# Autodesk Inventor assembly: Probe-clamp-v1
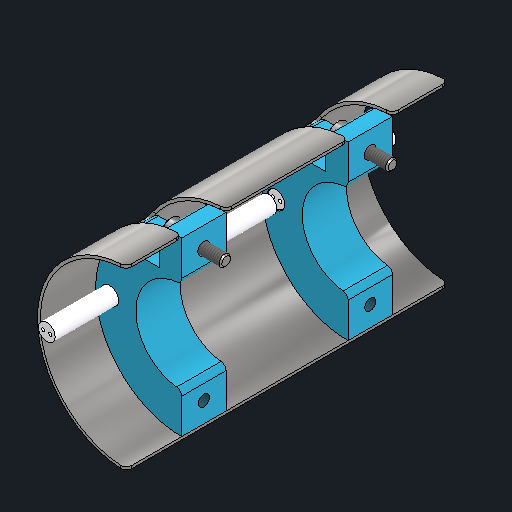
[picture p0: Inventor's stored thumbnail of the model, 512x512]
Saved by Autodesk Inventor 2026 (Build 300175050, 175E)
## iProperties
Created: 2024-06-05
Part Number: Probe-clamp-v1
Document SubType Name: Assembly
Designer: kuzmin
Author: kuzmin
## Documents named in this file (6)
- C:\Users\queez\Dropbox\Drawings\PIHTI\PALP\Probe-clamp-v1.iam
- C:\Users\queez\Dropbox\Drawings\PIHTI\PALP\WireHolderRing\WireHolderRing-ID16.4.ipt
- C:\Users\queez\Dropbox\Drawings\PIHTI\PALP\WireHolderRing.ipt
- C:\Users\queez\Dropbox\Drawings\PIHTI\ContentCenter\Fastners\M2x8-SHCS.ipt
- C:\Users\queez\Dropbox\Drawings\PIHTI\PALP\LP-screen-sheet-metal.ipt
- C:\Users\queez\Dropbox\Drawings\PIHTI\ContentCenter\Ceramics\Ceramic-tube-two-holes-phi3x0.5.ipt
## Components (8 placed, 4 different names)
1. WireHolderRing-ID16.4:2 — Mate:1, Flush:1, Mate:2, Mate:5
2. SS ISO 4762 M2 x 8:1
3. LP-screen-sheet-metal:1 — Mate:1, Flush:1, Mate:2, Mate:3, Mate:4, Flush:2
4. WireHolderRing-ID16.4:3 — Mate:3, Mate:4, Flush:2, Rigid:1, Mate:6, Mate:7
5. SS ISO 4762 M2 x 8:2 — Rigid:1
6. Ceramic-tube-two-holes-phi3x0.5:1 — Mate:5, Mate:8, Mate:9
7. Ceramic-tube-two-holes-phi3x0.5:2 — Mate:6, Mate:9
8. Ceramic-tube-two-holes-phi3x0.5:3 — Mate:7, Mate:8
## Relationships (13: Mate 9, Flush 2, RevoluteJoint 1, WeldJoint 1)
- [RevoluteJoint]: WireHolderRing-ID16.4:2 ↔ SS ISO 4762 M2 x 8:1
- Mate:1: WireHolderRing-ID16.4:2 ↔ LP-screen-sheet-metal:1
- Flush:1: WireHolderRing-ID16.4:2 ↔ LP-screen-sheet-metal:1
- Mate:2: WireHolderRing-ID16.4:2 ↔ LP-screen-sheet-metal:1
- Mate:3: LP-screen-sheet-metal:1 ↔ WireHolderRing-ID16.4:3
- Mate:4: LP-screen-sheet-metal:1 ↔ WireHolderRing-ID16.4:3
- Flush:2: LP-screen-sheet-metal:1 ↔ WireHolderRing-ID16.4:3
- Rigid:1 [WeldJoint]: WireHolderRing-ID16.4:3 ↔ SS ISO 4762 M2 x 8:2
- Mate:5: WireHolderRing-ID16.4:2 ↔ Ceramic-tube-two-holes-phi3x0.5:1
- Mate:6: WireHolderRing-ID16.4:3 ↔ Ceramic-tube-two-holes-phi3x0.5:2
- Mate:7: WireHolderRing-ID16.4:3 ↔ Ceramic-tube-two-holes-phi3x0.5:3
- Mate:8: Ceramic-tube-two-holes-phi3x0.5:1 ↔ Ceramic-tube-two-holes-phi3x0.5:3
- Mate:9: Ceramic-tube-two-holes-phi3x0.5:1 ↔ Ceramic-tube-two-holes-phi3x0.5:2
